# Autodesk Inventor assembly: wheelchair_secure_devices
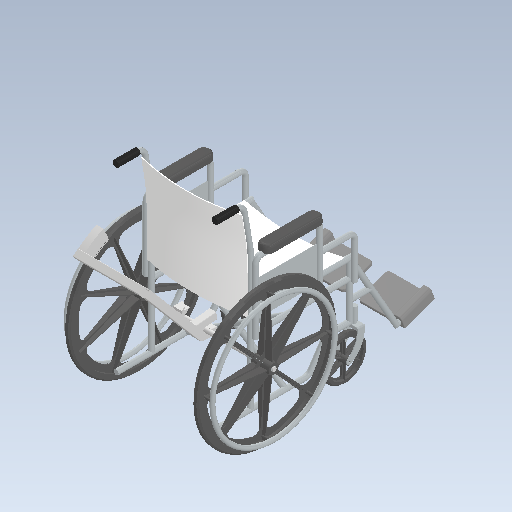
[picture p0: Inventor's stored thumbnail of the model, 512x512]
Saved by Autodesk Inventor 2021 (Build 250183000, 183)
## iProperties
Created: 2021-05-28
Part Number: wheelchair_secure_devices
Document SubType Name: Assembly
## Documents named in this file (7)
- C:\Users\ocon0143\OneDrive - Flinders\Advn Mech Design Shared\6_Development\2_Design\inventor\securing_mechanism\wheelchair_secure_devices.iam
- C:\Users\ocon0143\OneDrive - Flinders\Advn Mech Design Shared\6_Development\2_Design\inventor\securing_mechanism\secure_arm_holder.ipt
- C:\Users\ocon0143\OneDrive - Flinders\Advn Mech Design Shared\6_Development\2_Design\inventor\securing_mechanism\secure_wheel_bar.ipt
- C:\Users\ocon0143\OneDrive - Flinders\Advn Mech Design Shared\6_Development\2_Design\inventor\securing_mechanism\secure_width_bar.ipt
- C:\Users\ocon0143\OneDrive - Flinders\Advn Mech Design Shared\6_Development\2_Design\inventor\vehicle_wheelchair\wheelchair\wheelchair.ipt
- C:\Users\ocon0143\OneDrive - Flinders\Advn Mech Design Shared\6_Development\2_Design\inventor\securing_mechanism\axle_example.ipt
- C:\Users\ocon0143\OneDrive - Flinders\Advn Mech Design Shared\6_Development\2_Design\inventor\securing_mechanism\secure_to_hoop_machined.ipt
## Components (6 placed, 6 different names)
1. secure_arm_holder:1 — Mate:2, Mate:3, Flush:3, Flush:5, Mate:6, Flush:6, Mate:7
2. secure_wheel_bar:1 — Mate:4, Flush:4, Mate:8
3. secure_width_bar:1 — Mate:3, Flush:3, Mate:4, Flush:4, Flush:5, Mate:8
4. wheelchair:1 — Mate:1, Flush:1
5. axle_example:1 — Mate:1, Flush:2, Mate:2
6. secure_to_hoop_machined:1 — Mate:6, Flush:6, Mate:7
## Relationships (13: Mate 7, Flush 6)
- Mate:1: wheelchair:1 ↔ axle_example:1
- Flush:1 (220 mm): wheelchair:1
- Flush:2: axle_example:1
- Mate:2: secure_arm_holder:1 ↔ axle_example:1
- Mate:3: secure_arm_holder:1 ↔ secure_width_bar:1
- Flush:3: secure_arm_holder:1 ↔ secure_width_bar:1
- Mate:4: secure_wheel_bar:1 ↔ secure_width_bar:1
- Flush:4: secure_wheel_bar:1 ↔ secure_width_bar:1
- Flush:5: secure_arm_holder:1 ↔ secure_width_bar:1
- Mate:6: secure_arm_holder:1 ↔ secure_to_hoop_machined:1
- Flush:6: secure_arm_holder:1 ↔ secure_to_hoop_machined:1
- Mate:7: secure_arm_holder:1 ↔ secure_to_hoop_machined:1
- Mate:8: secure_wheel_bar:1 ↔ secure_width_bar:1
